# Autodesk Inventor assembly: 108 Pasador-Traba Resorte
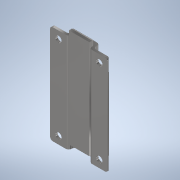
[picture p0: Inventor's stored thumbnail of the model, 180x180]
Saved by Autodesk Inventor 2021.2 (Build 252289000, 289)
## iProperties
Created: 2026-08-24
Part Number: 108 Pasador-Traba Resorte
Document SubType Name: Assembly
Designer: nelso
Author: nelso
## Documents named in this file (3)
- C:\Users\nelso\Desktop\Soporte-Paciente-Espinografia\Workspace\108 Pasador-Traba Resorte.iam
- C:\Users\nelso\Desktop\Soporte-Paciente-Espinografia\Workspace\Pieza1 Pasador.ipt
- C:\Users\nelso\Desktop\Soporte-Paciente-Espinografia\Workspace\Pieza2 Pasador.ipt
## Components (2 placed, 2 different names)
1. Pieza1 Pasador:1 — Mate:1, Mate:2
2. Pieza2 Pasador:1 — Mate:1, Mate:2, Mate:3, Mate:4, Flush:1
## Relationships (5: Mate 4, Flush 1)
- Mate:1: Pieza1 Pasador:1 ↔ Pieza2 Pasador:1
- Mate:2: Pieza1 Pasador:1 ↔ Pieza2 Pasador:1
- Mate:3: Pieza2 Pasador:1
- Mate:4: Pieza2 Pasador:1
- Flush:1: Pieza2 Pasador:1
